# Autodesk Inventor assembly: assm
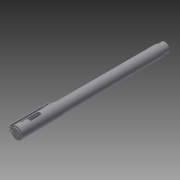
[picture p0: Inventor's stored thumbnail of the model, 180x180]
Saved by Autodesk Inventor 2015 (Build 190159000, 159)
## iProperties
Created: 2014-11-30
Part Number: assm
Document SubType Name: Assembly
Designer: zenkr
Author: zenkr
## Documents named in this file (8)
- D:\z\zenkr\design model\pen\assm.iam
- D:\z\zenkr\design model\pen\body.ipt
- D:\z\zenkr\design model\pen\backtop.ipt
- D:\z\zenkr\design model\pen\conver.ipt
- D:\z\zenkr\design model\pen\coverbody.ipt
- D:\z\zenkr\design model\pen\snip.ipt
- D:\z\zenkr\design model\pen\toptube.ipt
- D:\z\zenkr\design model\pen\top.ipt
## Components (7 placed, 7 different names)
1. body:1 — 配合:1, 配合:2, 配合:3, 配合:4, 配合:6, 配合:7, 配合:13
2. backtop:1 — 配合:1, 配合:2
3. conver:1 — 配合:3, 配合:4, 配合:11, 表面齐平:1
4. coverbody:1 — 配合:6, 配合:7, 配合:8, 配合:9, 配合:10, 配合:13
5. snip:1 — 配合:8, 配合:9, 配合:10
6. toptube:1 — 配合:11, 表面齐平:1, 配合:12, 表面齐平:2
7. top:1 — 配合:12, 表面齐平:2
## Relationships (14: Mate 12, Flush 2)
- 配合:1 [Mate]: body:1 ↔ backtop:1
- 配合:2 [Mate]: body:1 ↔ backtop:1
- 配合:3 [Mate]: body:1 ↔ conver:1
- 配合:4 [Mate]: body:1 ↔ conver:1
- 配合:6 [Mate]: body:1 ↔ coverbody:1
- 配合:7 [Mate]: body:1 ↔ coverbody:1
- 配合:8 [Mate]: coverbody:1 ↔ snip:1
- 配合:9 [Mate]: coverbody:1 ↔ snip:1
- 配合:10 [Mate]: coverbody:1 ↔ snip:1
- 配合:11 [Mate]: conver:1 ↔ toptube:1
- 表面齐平:1 [Flush] (-3 mm): conver:1 ↔ toptube:1
- 配合:12 [Mate]: toptube:1 ↔ top:1
- 表面齐平:2 [Flush] (-0.8 mm): toptube:1 ↔ top:1
- 配合:13 [Mate]: body:1 ↔ coverbody:1
